# Autodesk Inventor assembly: capcule_assenbly
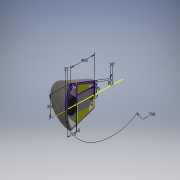
[picture p0: Inventor's stored thumbnail of the model, 180x180]
Saved by Autodesk Inventor 2019.3 (Build 233278000, 278)
## iProperties
Created: 2019-01-10
Part Number: capcule_assenbly
Material: 一般
Document SubType Name: Assembly
Designer: masaya
Author: masaya
## Documents named in this file (6)
- D:\Documents\卒業設計\seed_bank_in_space\cad\capcule\capcule_assenbly.iam
- D:\Documents\卒業設計\seed_bank_in_space\cad\capcule\hakoooo.ipt
- D:\Documents\卒業設計\seed_bank_in_space\cad\capcule\parachute.ipt
- D:\Documents\卒業設計\seed_bank_in_space\cad\capcule\seed_in_alm.ipt
- D:\Documents\卒業設計\seed_bank_in_space\cad\capcule\tank.ipt
- D:\Documents\卒業設計\seed_bank_in_space\cad\capcule\abionics.ipt
## Components (6 placed, 5 different names)
1. hakoooo:1 — メイト:1, フラッシュ:1, 正接:1, メイト:2, フラッシュ:2, 正接:2, 正接:3, フラッシュ:3, フラッシュ:4, フラッシュ:5, フラッシュ:6, メイト:3
2. parachute:1 — メイト:1, フラッシュ:1, 正接:1
3. seed_in_alm:1 — メイト:2, フラッシュ:2, 正接:2
4. tank:1 — 正接:3, フラッシュ:3, 正接:4, 対称度:1
5. tank:2 — 対称度:1, フラッシュ:5
6. abionics:1 — フラッシュ:6, メイト:3
## Relationships (14: Flush 6, Tangent 4, Mate 3, Symmetry 1)
- メイト:1 [Mate]: hakoooo:1 ↔ parachute:1
- フラッシュ:1 [Flush]: hakoooo:1 ↔ parachute:1
- 正接:1 [Tangent]: hakoooo:1 ↔ parachute:1
- メイト:2 [Mate]: hakoooo:1 ↔ seed_in_alm:1
- フラッシュ:2 [Flush]: hakoooo:1 ↔ seed_in_alm:1
- 正接:2 [Tangent]: hakoooo:1 ↔ seed_in_alm:1
- 正接:3 [Tangent]: hakoooo:1 ↔ tank:1
- フラッシュ:3 [Flush]: hakoooo:1 ↔ tank:1
- フラッシュ:4 [Flush]: hakoooo:1
- 正接:4 [Tangent]: tank:1
- 対称度:1 [Symmetry]: tank:1 ↔ tank:2
- フラッシュ:5 [Flush]: hakoooo:1 ↔ tank:2
- フラッシュ:6 [Flush]: hakoooo:1 ↔ abionics:1
- メイト:3 [Mate]: hakoooo:1 ↔ abionics:1
